# Autodesk Inventor assembly: Setup_1
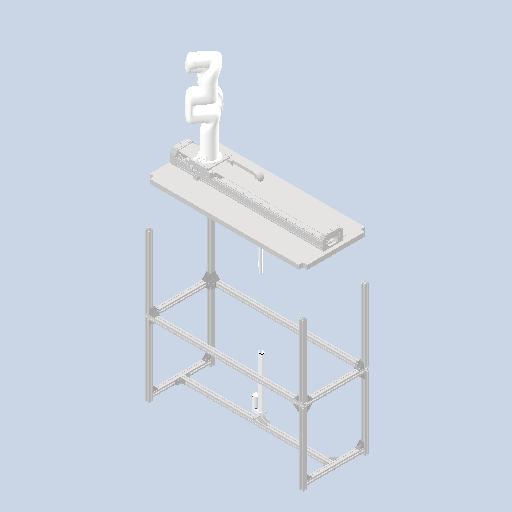
[picture p0: Inventor's stored thumbnail of the model, 512x512]
Saved by Autodesk Inventor 2025 (Build 290162000, 162)
## iProperties
Created: 2024-06-18
Part Number: Setup_1
Document SubType Name: Assembly
Designer: User
Author: User
## Documents named in this file (14)
- C:\Users\User\OneDrive\Documents\FYP\Inventor_Designs\Setup_1.iam
- C:\Users\User\OneDrive\Documents\FYP\Inventor_Designs\Metal Profile\Metal Profile 110 cm.ipt
- C:\Users\User\OneDrive\Documents\FYP\Inventor_Designs\Metal Profile\Metal Profile 40 cm.ipt
- C:\Users\User\OneDrive\Documents\FYP\Inventor_Designs\Metal Profile\Metal Profile 50 cm.ipt
- C:\Users\User\OneDrive\Documents\FYP\Inventor_Designs\Metal Profile\Metal Profile 104 cm.ipt
- C:\Users\User\OneDrive\Documents\FYP\Inventor_Designs\Linear Motor\Motor.ipt
- C:\Users\User\OneDrive\Documents\FYP\Inventor_Designs\Designs_Arm\Platform.ipt
- C:\Users\User\OneDrive\Documents\FYP\Inventor_Designs\Platform\Platform_Arm.ipt
- C:\Users\User\OneDrive\Documents\FYP\Inventor_Designs\Designs_Arm\Arm.iam
- C:\Users\User\OneDrive\Documents\FYP\Inventor_Designs\Linear Actuator\300mm Body.ipt
- C:\Users\User\OneDrive\Documents\FYP\Inventor_Designs\Linear Actuator\300mm Rod.ipt
- C:\Users\User\OneDrive\Documents\FYP\Inventor_Designs\Triangle Bracket\Triangle Bracket.ipt
- C:\Users\User\OneDrive\Documents\FYP\Inventor_Designs\Clevis Pin\Celvis Pin.ipt
- C:\Users\User\OneDrive\Documents\FYP\Inventor_Designs\L Bracket\L Angle Bracket 30x30.ipt
## Components (53 placed, 13 different names)
1. Metal Profile 110 cm:1 — Mate:1, Mate:3, Flush:1, Mate:4, Flush:3, Mate:6, Mate:7, Mate:8, Flush:5, Mate:15, Mate:16, Mate:17, Mate:57, Mate:58, Mate:94, Mate:98, Mate:106, Mate:108, Mate:122, Mate:127
2. Metal Profile 40 cm:2 — Mate:1, Mate:2, Mate:3, Flush:1, Flush:2, Flush:3, Mate:6, Mate:23, Mate:95, Mate:96, Mate:109, Mate:111, Mate:124, Mate:126
3. Metal Profile 110 cm:2 — Mate:2, Flush:2, Mate:5, Flush:4, Mate:9, Mate:10, Mate:11, Mate:12, Mate:13, Mate:14, Mate:47, Mate:56, Mate:61, Mate:97, Mate:100, Mate:102, Mate:103, Mate:116, Mate:128
4. Metal Profile 40 cm:3 — Mate:4, Mate:5, Flush:4, Mate:20, Mate:99, Mate:101, Mate:112, Mate:114, Mate:117, Mate:120
5. Metal Profile 50 cm:1 — Mate:7, Mate:8, Flush:5, Mate:22, Mate:50, Mate:51, Mate:87, Mate:107
6. Metal Profile 50 cm:2 — Mate:9, Mate:10, Mate:11, Mate:21, Mate:48, Mate:49, Mate:90, Mate:91, Flush:11, Mate:110
7. Metal Profile 50 cm:3 — Mate:15, Mate:16, Mate:17, Mate:18, Mate:52, Mate:53, Mate:80, Mate:105
8. Metal Profile 50 cm:4 — Mate:12, Mate:13, Mate:14, Mate:19, Mate:54, Mate:55, Mate:93, Mate:104, Mate:113
9. Metal Profile 40 cm:4 — Mate:18, Mate:19, Mate:20, Mate:59, Mate:60, Mate:79, Mate:83, Mate:85, Mate:92
10. Metal Profile 40 cm:5 — Mate:21, Mate:22, Mate:23, Flush:9, Mate:78, Mate:81, Mate:88, Mate:89
11. Metal Profile 50 cm:5 — Mate:50, Mate:51, Mate:58, Mate:125, Mate:130
12. Metal Profile 50 cm:6 — Mate:47, Mate:48, Mate:49, Mate:123, Mate:129
13. Metal Profile 50 cm:7 — Mate:52, Mate:53, Mate:57, Mate:73, Mate:119, Mate:121
14. Metal Profile 50 cm:8 — Mate:54, Mate:55, Mate:56, Mate:62, Mate:63, Mate:115, Mate:118
15. Metal Profile 104 cm:1 — Mate:59, Mate:60, Mate:61, Mate:69, Flush:8, Mate:77, Mate:82, Mate:84, Mate:86
16. Motor:1 — Mate:64, Flush:6, Flush:7, Mate:65, Mate:66, Mate:67
17. Platform:1
18. Platform_Arm:1 — Mate:62, Mate:63, Mate:64, Flush:6, Flush:7, Mate:72, Flush:10
19. Arm:1 [sub-assembly] — Mate:65, Mate:66, Mate:67
20. Triangle Bracket:1 — Mate:69, Flush:8, Flush:9, Insert:1, Mate:71
21. 300mm Body:1 — Insert:1, Mate:74
22. Celvis Pin:1 — Mate:71
23. Triangle Bracket:2 — Mate:72, Flush:10, Mate:73, Mate:75
24. 300mm Rod:1 — Mate:74, Mate:75, Mate:76
25. Celvis Pin:2 — Mate:76
26. L Angle Bracket 30x30:1 — Mate:107, Mate:108
27. L Angle Bracket 30x30:2 — Mate:96, Mate:97
28. L Angle Bracket 30x30:3 — Mate:94, Mate:95
29. L Angle Bracket 30x30:4 — Mate:77, Mate:78
30. L Angle Bracket 30x30:5 — Mate:103, Mate:104
31. L Angle Bracket 30x30:6 — Mate:118, Mate:117
32. L Angle Bracket 30x30:7 — Mate:113, Mate:114
33. L Angle Bracket 30x30:8 — Mate:110, Mate:111
34. L Angle Bracket 30x30:9 — Mate:112
35. L Angle Bracket 30x30:10 — Mate:109
36. L Angle Bracket 30x30:11 — Mate:102, Flush:11
37. L Angle Bracket 30x30:12 — Mate:89, Mate:90, Mate:91
38. L Angle Bracket 30x30:13 — Mate:98, Mate:99
39. L Angle Bracket 30x30:14 — Mate:87, Mate:88
40. L Angle Bracket 30x30:15 — Mate:85, Mate:86
41. L Angle Bracket 30x30:16 — Mate:100, Mate:101
42. L Angle Bracket 30x30:17 — Mate:92, Mate:93
43. L Angle Bracket 30x30:18 — Mate:83, Mate:84
44. L Angle Bracket 30x30:19 — Mate:79, Mate:80
45. L Angle Bracket 30x30:20 — Mate:81, Mate:82
46. L Angle Bracket 30x30:21 — Mate:119, Mate:120
47. L Angle Bracket 30x30:23 — Mate:105, Mate:106
48. L Angle Bracket 30x30:24 — Mate:115, Mate:116
49. L Angle Bracket 30x30:28 — Mate:123, Mate:124
50. L Angle Bracket 30x30:29 — Mate:125, Mate:126
51. L Angle Bracket 30x30:30 — Mate:128, Mate:129
52. L Angle Bracket 30x30:32 — Mate:121, Mate:122
53. L Angle Bracket 30x30:33 — Mate:127, Mate:130
## Relationships (117: Mate 105, Flush 11, Insert 1)
- Mate:1: Metal Profile 110 cm:1 ↔ Metal Profile 40 cm:2
- Mate:2: Metal Profile 40 cm:2 ↔ Metal Profile 110 cm:2
- Mate:3: Metal Profile 110 cm:1 ↔ Metal Profile 40 cm:2
- Flush:1: Metal Profile 110 cm:1 ↔ Metal Profile 40 cm:2
- Flush:2: Metal Profile 40 cm:2 ↔ Metal Profile 110 cm:2
- Mate:4: Metal Profile 110 cm:1 ↔ Metal Profile 40 cm:3
- Flush:3: Metal Profile 110 cm:1 ↔ Metal Profile 40 cm:2
- Mate:5: Metal Profile 110 cm:2 ↔ Metal Profile 40 cm:3
- Flush:4: Metal Profile 110 cm:2 ↔ Metal Profile 40 cm:3
- Mate:6: Metal Profile 110 cm:1 ↔ Metal Profile 40 cm:2
- Mate:7: Metal Profile 110 cm:1 ↔ Metal Profile 50 cm:1
- Mate:8: Metal Profile 110 cm:1 ↔ Metal Profile 50 cm:1
- Flush:5: Metal Profile 110 cm:1 ↔ Metal Profile 50 cm:1
- Mate:9: Metal Profile 110 cm:2 ↔ Metal Profile 50 cm:2
- Mate:10: Metal Profile 110 cm:2 ↔ Metal Profile 50 cm:2
- Mate:11: Metal Profile 110 cm:2 ↔ Metal Profile 50 cm:2
- Mate:12: Metal Profile 110 cm:2 ↔ Metal Profile 50 cm:4
- Mate:13: Metal Profile 110 cm:2 ↔ Metal Profile 50 cm:4
- Mate:14: Metal Profile 110 cm:2 ↔ Metal Profile 50 cm:4
- Mate:15: Metal Profile 110 cm:1 ↔ Metal Profile 50 cm:3
- Mate:16: Metal Profile 110 cm:1 ↔ Metal Profile 50 cm:3
- Mate:17: Metal Profile 110 cm:1 ↔ Metal Profile 50 cm:3
- Mate:18: Metal Profile 50 cm:3 ↔ Metal Profile 40 cm:4
- Mate:19: Metal Profile 50 cm:4 ↔ Metal Profile 40 cm:4
- Mate:20 (450 mm): Metal Profile 40 cm:3 ↔ Metal Profile 40 cm:4
- Mate:21: Metal Profile 50 cm:2 ↔ Metal Profile 40 cm:5
- Mate:22: Metal Profile 50 cm:1 ↔ Metal Profile 40 cm:5
- Mate:23 (450 mm): Metal Profile 40 cm:2 ↔ Metal Profile 40 cm:5
- Mate:47: Metal Profile 110 cm:2 ↔ Metal Profile 50 cm:6
- Mate:48: Metal Profile 50 cm:2 ↔ Metal Profile 50 cm:6
- Mate:49: Metal Profile 50 cm:2 ↔ Metal Profile 50 cm:6
- Mate:50: Metal Profile 50 cm:1 ↔ Metal Profile 50 cm:5
- Mate:51: Metal Profile 50 cm:1 ↔ Metal Profile 50 cm:5
- Mate:52: Metal Profile 50 cm:3 ↔ Metal Profile 50 cm:7
- Mate:53: Metal Profile 50 cm:3 ↔ Metal Profile 50 cm:7
- Mate:54: Metal Profile 50 cm:4 ↔ Metal Profile 50 cm:8
- Mate:55: Metal Profile 50 cm:4 ↔ Metal Profile 50 cm:8
- Mate:56: Metal Profile 110 cm:2 ↔ Metal Profile 50 cm:8
- Mate:57: Metal Profile 110 cm:1 ↔ Metal Profile 50 cm:7
- Mate:58: Metal Profile 110 cm:1 ↔ Metal Profile 50 cm:5
- Mate:59 (185 mm): Metal Profile 40 cm:4 ↔ Metal Profile 104 cm:1
- Mate:60: Metal Profile 40 cm:4 ↔ Metal Profile 104 cm:1
- Mate:61 (499 mm): Metal Profile 110 cm:2 ↔ Metal Profile 104 cm:1
- Mate:62: Metal Profile 50 cm:8 ↔ Platform_Arm:1
- Mate:63: Metal Profile 50 cm:8 ↔ Platform_Arm:1
- Mate:64: Motor:1 ↔ Platform_Arm:1
- Flush:6 (20 mm): Motor:1 ↔ Platform_Arm:1
- Flush:7 (160 mm): Motor:1 ↔ Platform_Arm:1
- Mate:65: Motor:1 ↔ Arm:1
- Mate:66: Motor:1 ↔ Arm:1
- Mate:67: Motor:1 ↔ Arm:1
- Mate:69: Metal Profile 104 cm:1 ↔ Triangle Bracket:1
- Flush:8 (2 mm): Metal Profile 104 cm:1 ↔ Triangle Bracket:1
- Flush:9 (570 mm): Metal Profile 40 cm:5 ↔ Triangle Bracket:1
- Insert:1 (-22 mm): Triangle Bracket:1 ↔ 300mm Body:1
- Mate:71: Triangle Bracket:1 ↔ Celvis Pin:1
- Mate:72: Platform_Arm:1 ↔ Triangle Bracket:2
- Flush:10 (570 mm): Platform_Arm:1 ↔ Triangle Bracket:2
- Mate:73 (187 mm): Metal Profile 50 cm:7 ↔ Triangle Bracket:2
- Mate:74: 300mm Body:1 ↔ 300mm Rod:1
- Mate:75: Triangle Bracket:2 ↔ 300mm Rod:1
- Mate:76: 300mm Rod:1 ↔ Celvis Pin:2
- Mate:77: Metal Profile 104 cm:1 ↔ L Angle Bracket 30x30:4
- Mate:78: Metal Profile 40 cm:5 ↔ L Angle Bracket 30x30:4
- Mate:79: Metal Profile 40 cm:4 ↔ L Angle Bracket 30x30:19
- Mate:80: Metal Profile 50 cm:3 ↔ L Angle Bracket 30x30:19
- Mate:81: Metal Profile 40 cm:5 ↔ L Angle Bracket 30x30:20
- Mate:82: Metal Profile 104 cm:1 ↔ L Angle Bracket 30x30:20
- Mate:83: Metal Profile 40 cm:4 ↔ L Angle Bracket 30x30:18
- Mate:84: Metal Profile 104 cm:1 ↔ L Angle Bracket 30x30:18
- Mate:85: Metal Profile 40 cm:4 ↔ L Angle Bracket 30x30:15
- Mate:86: Metal Profile 104 cm:1 ↔ L Angle Bracket 30x30:15
- Mate:87: Metal Profile 50 cm:1 ↔ L Angle Bracket 30x30:14
- Mate:88: Metal Profile 40 cm:5 ↔ L Angle Bracket 30x30:14
- Mate:89: Metal Profile 40 cm:5 ↔ L Angle Bracket 30x30:12
- Mate:90: Metal Profile 50 cm:2 ↔ L Angle Bracket 30x30:12
- Mate:91: Metal Profile 50 cm:2 ↔ L Angle Bracket 30x30:12
- Mate:92: Metal Profile 40 cm:4 ↔ L Angle Bracket 30x30:17
- Mate:93: Metal Profile 50 cm:4 ↔ L Angle Bracket 30x30:17
- Mate:94: Metal Profile 110 cm:1 ↔ L Angle Bracket 30x30:3
- Mate:95: Metal Profile 40 cm:2 ↔ L Angle Bracket 30x30:3
- Mate:96: Metal Profile 40 cm:2 ↔ L Angle Bracket 30x30:2
- Mate:97: Metal Profile 110 cm:2 ↔ L Angle Bracket 30x30:2
- Mate:98: Metal Profile 110 cm:1 ↔ L Angle Bracket 30x30:13
- Mate:99: Metal Profile 40 cm:3 ↔ L Angle Bracket 30x30:13
- Mate:100: Metal Profile 110 cm:2 ↔ L Angle Bracket 30x30:16
- Mate:101: Metal Profile 40 cm:3 ↔ L Angle Bracket 30x30:16
- Mate:102: Metal Profile 110 cm:2 ↔ L Angle Bracket 30x30:11
- Mate:103: Metal Profile 110 cm:2 ↔ L Angle Bracket 30x30:5
- Flush:11: Metal Profile 50 cm:2 ↔ L Angle Bracket 30x30:11
- Mate:104: Metal Profile 50 cm:4 ↔ L Angle Bracket 30x30:5
- Mate:105: Metal Profile 50 cm:3 ↔ L Angle Bracket 30x30:23
- Mate:106: Metal Profile 110 cm:1 ↔ L Angle Bracket 30x30:23
- Mate:107: Metal Profile 50 cm:1 ↔ L Angle Bracket 30x30:1
- Mate:108: Metal Profile 110 cm:1 ↔ L Angle Bracket 30x30:1
- Mate:109: Metal Profile 40 cm:2 ↔ L Angle Bracket 30x30:10
- Mate:110: Metal Profile 50 cm:2 ↔ L Angle Bracket 30x30:8
- Mate:111: Metal Profile 40 cm:2 ↔ L Angle Bracket 30x30:8
- Mate:112: Metal Profile 40 cm:3 ↔ L Angle Bracket 30x30:9
- Mate:113: Metal Profile 50 cm:4 ↔ L Angle Bracket 30x30:7
- Mate:114: Metal Profile 40 cm:3 ↔ L Angle Bracket 30x30:7
- Mate:115: Metal Profile 50 cm:8 ↔ L Angle Bracket 30x30:24
- Mate:118: Metal Profile 50 cm:8 ↔ L Angle Bracket 30x30:6
- Mate:116: Metal Profile 110 cm:2 ↔ L Angle Bracket 30x30:24
- Mate:117: Metal Profile 40 cm:3 ↔ L Angle Bracket 30x30:6
- Mate:119: Metal Profile 50 cm:7 ↔ L Angle Bracket 30x30:21
- Mate:120: Metal Profile 40 cm:3 ↔ L Angle Bracket 30x30:21
- Mate:121: Metal Profile 50 cm:7 ↔ L Angle Bracket 30x30:32
- Mate:122: Metal Profile 110 cm:1 ↔ L Angle Bracket 30x30:32
- Mate:123: Metal Profile 50 cm:6 ↔ L Angle Bracket 30x30:28
- Mate:124: Metal Profile 40 cm:2 ↔ L Angle Bracket 30x30:28
- Mate:125: Metal Profile 50 cm:5 ↔ L Angle Bracket 30x30:29
- Mate:126: Metal Profile 40 cm:2 ↔ L Angle Bracket 30x30:29
- Mate:127: Metal Profile 110 cm:1 ↔ L Angle Bracket 30x30:33
- Mate:128: Metal Profile 110 cm:2 ↔ L Angle Bracket 30x30:30
- Mate:129: Metal Profile 50 cm:6 ↔ L Angle Bracket 30x30:30
- Mate:130: Metal Profile 50 cm:5 ↔ L Angle Bracket 30x30:33
